# Autodesk Inventor assembly: LAPTOP
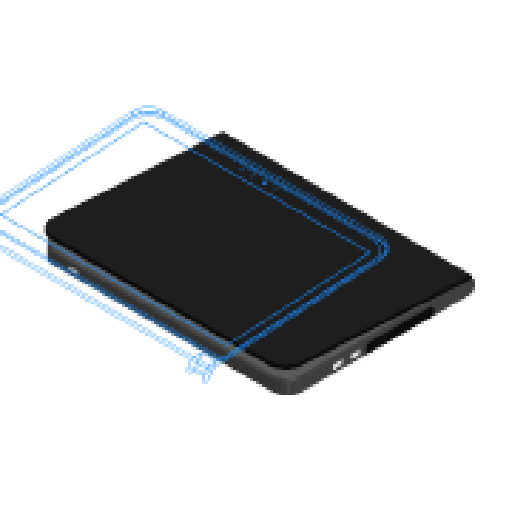
[picture p0: Inventor's stored thumbnail of the model, 512x512]
Saved by Autodesk Inventor 2025 (Build 290162000, 162)
## iProperties
Created: 2017-02-18
Part Number: LAPTOP
Document SubType Name: Assembly
Designer: Ali
Author: Ali
## Documents named in this file (4)
- C:\Users\derm\Desktop\puppycat\LAPTOP.iam
- C:\Users\derm\Desktop\puppycat\BOARD.ipt
- C:\Users\derm\Desktop\puppycat\KEYBOARD.ipt
- C:\Users\derm\Desktop\puppycat\MONITOR.ipt
## Components (3 placed, 3 different names)
1. BOARD:1 — Flush:2, Mate:1, Mate:2
2. KEYBOARD:1 — Flush:2
3. MONITOR:1 — Mate:1, Mate:2
## Relationships (3: Mate 2, Flush 1)
- Flush:2: BOARD:1 ↔ KEYBOARD:1
- Mate:1: BOARD:1 ↔ MONITOR:1
- Mate:2: BOARD:1 ↔ MONITOR:1
